# Autodesk Inventor assembly: final_assembly_2017_SuperUltraLow
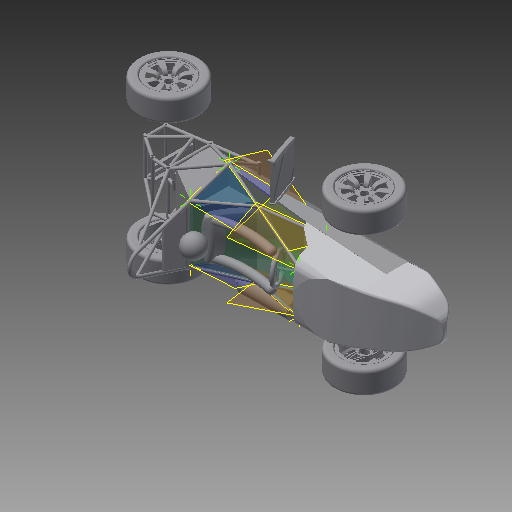
[picture p0: Inventor's stored thumbnail of the model, 512x512]
Saved by Autodesk Inventor 2018.2 (Build 222227000, 227)
## iProperties
Created: 2017-10-13
Part Number: final_assembly_2017_SuperUltraLow
Material: 一般
Document SubType Name: Assembly
Designer: kuwano
Sending System: Autodesk Inventor 2018
Preprocessor: ST-DEVELOPER v16.13
Title: D:\kuwano\Documents\Inventor\KITformula\CFD_KS-14\KS-14\stl\final_assembly_2017_SuperUltraLow.stp
Author: kuwano
## Documents named in this file (15)
- Z:\各班フォルダ\2018\ボディ\カウル\AeroCAD2018\CAD\Inventor\Assembly(KS-14.ver)\KS-14_SLow\KS-14_SLow.iam
- Z:\各班フォルダ\2018\ボディ\カウル\AeroCAD2018\CAD\Inventor\Assembly(KS-14.ver)\KS-14_SLow\parts\parts\frame3kaiseki_retutch.ipt
- Z:\各班フォルダ\2018\ボディ\カウル\AeroCAD2018\CAD\Inventor\Assembly(KS-14.ver)\KS-14_SLow\parts\parts\F-Upright.iam
- Z:\各班フォルダ\2018\ボディ\カウル\AeroCAD2018\CAD\Inventor\Assembly(KS-14.ver)\KS-14_SLow\parts\parts\R-Upright.iam
- Z:\各班フォルダ\2018\ボディ\カウル\AeroCAD2018\CAD\Inventor\Assembly(KS-14.ver)\KS-14_SLow\parts\parts\driver.ipt
- Z:\各班フォルダ\2018\ボディ\カウル\AeroCAD2018\CAD\Inventor\Assembly(KS-14.ver)\KS-14_SLow\parts\parts\steering assembly.iam
- Z:\各班フォルダ\2018\ボディ\カウル\AeroCAD2018\CAD\Inventor\Assembly(KS-14.ver)\KS-14_SLow\parts\parts\F-Upright_MIR1.iam
- Z:\各班フォルダ\2018\ボディ\カウル\AeroCAD2018\CAD\Inventor\Assembly(KS-14.ver)\KS-14_SLow\parts\parts\R-Upright_MIR2.iam
- Z:\各班フォルダ\2018\ボディ\カウル\AeroCAD2018\CAD\Inventor\Assembly(KS-14.ver)\KS-14_SLow\parts\parts\2017 exhaust assembly_retouch.ipt
- Z:\各班フォルダ\2018\ボディ\カウル\AeroCAD2018\CAD\Inventor\Assembly(KS-14.ver)\KS-14_SLow\parts\parts\kaul_reretouch.ipt
- Z:\各班フォルダ\2018\ボディ\カウル\AeroCAD2018\CAD\Inventor\Assembly(KS-14.ver)\KS-14_SLow\parts\parts\newbody.ipt
- Z:\各班フォルダ\2018\ボディ\カウル\AeroCAD2018\CAD\Inventor\Assembly(KS-14.ver)\KS-14_SLow\parts\parts\wall.ipt
- Z:\各班フォルダ\2018\ボディ\カウル\AeroCAD2018\CAD\Inventor\Assembly(KS-14.ver)\KS-14_SLow\parts\parts\wall_MIR1.ipt
- Z:\各班フォルダ\2018\ボディ\カウル\AeroCAD2018\CAD\Inventor\Assembly(KS-14.ver)\KS-14_SLow\parts\parts\2015Wheel watanabe.ipt
- Z:\各班フォルダ\2018\ボディ\カウル\AeroCAD2018\CAD\Inventor\Assembly(KS-14.ver)\KS-14_SLow\parts\parts\radiator 2014 kaiseki_re.ipt
## Components (17 placed, 14 different names)
1. frame3kaiseki_retutch:1 — メイト:2, メイト:3, メイト:4, メイト:5, メイト:6
2. F-Upright:1 [sub-assembly]
3. R-Upright:1 [sub-assembly]
4. driver:1
5. steering assembly:1 [sub-assembly]
6. F-Upright_MIR1:1 [sub-assembly]
7. R-Upright_MIR2:1 [sub-assembly]
8. 2017 exhaust assembly_retouch:1
9. kaul_reretouch:1 — メイト:1
10. newbody:1 — メイト:1
11. wall:1 — フラッシュ:1, フラッシュ:2, フラッシュ:3, メイト:2, メイト:3, メイト:4, メイト:5, メイト:6
12. wall_MIR1:1 — メイト:7, メイト:8, フラッシュ:4
13. 2015Wheel watanabe:1
14. 2015Wheel watanabe:2
15. 2015Wheel watanabe:3
16. 2015Wheel watanabe:4
17. radiator 2014 kaiseki_re:1
## Relationships (12: Mate 8, Flush 4)
- メイト:1 [Mate]: kaul_reretouch:1 ↔ newbody:1
- フラッシュ:1 [Flush]: wall:1
- フラッシュ:2 [Flush]: wall:1
- フラッシュ:3 [Flush]: wall:1
- メイト:2 [Mate]: frame3kaiseki_retutch:1 ↔ wall:1
- メイト:3 [Mate]: frame3kaiseki_retutch:1 ↔ wall:1
- メイト:4 [Mate]: frame3kaiseki_retutch:1 ↔ wall:1
- メイト:5 [Mate]: frame3kaiseki_retutch:1 ↔ wall:1
- メイト:6 [Mate]: frame3kaiseki_retutch:1 ↔ wall:1
- メイト:7 [Mate]: wall_MIR1:1
- メイト:8 [Mate]: wall_MIR1:1
- フラッシュ:4 [Flush]: wall_MIR1:1
